# Autodesk Inventor assembly: axis5_6  compact
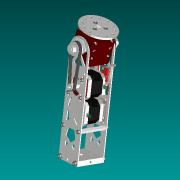
[picture p0: Inventor's stored thumbnail of the model, 180x180]
Saved by Autodesk Inventor 2020 (Build 240168000, 168)
## iProperties
Created: 2020-05-15
Part Number: axis5_6  compact
Document SubType Name: Assembly
Designer: stefa
Author: stefa
## Documents named in this file (21)
- D:\github_gedeeld\BeerMinder\3D-model\axis5_6\axis5_6  compact.iam
- D:\github_gedeeld\BeerMinder\3D-model\pulleys\GT2 Timing Pulley 36T - 8mm as.ipt
- D:\github_gedeeld\BeerMinder\3D-model\stepper motors\42BYG Stepper Motor.ipt
- D:\github_gedeeld\BeerMinder\3D-model\pulleys\GT2 Pulley 16T - 5mm as.ipt
- D:\github_gedeeld\BeerMinder\3D-model\axis5_6\bovenarm - links.ipt
- D:\github_gedeeld\BeerMinder\3D-model\bearings\lager 8mm - buiten 14 (sven 2 stuks).ipt
- D:\github_gedeeld\BeerMinder\3D-model\axis5_6\differential gearbox compact.iam
- D:\github_gedeeld\BeerMinder\3D-model\pulleys\tandriem32Tnaar16T_lengte280.ipt
- D:\github_gedeeld\BeerMinder\3D-model\pulleys\tandriem32Tnaar16T_lengte188.ipt
- D:\github_gedeeld\BeerMinder\3D-model\axis5_6\bovenarm - rechts.ipt
- D:\github_gedeeld\BeerMinder\3D-model\axis5_6\vul as platen.ipt
- D:\github_gedeeld\BeerMinder\3D-model\axis5_6\upvulling steppers axis5_6.ipt
- D:\github_gedeeld\BeerMinder\3D-model\boutjesEnMoertjes\ISO 4762 - M4 x 16ISO.ipt
- C:\Users\stefa\Documents\Inventor\Content Center Files\R2020\en-US\ISO 7089\ISO 7089 - 3 - 140 HV(1).ipt
- D:\github_gedeeld\BeerMinder\3D-model\axis5_6\bevestegingsKoppeling axis4_5.ipt
- C:\Users\stefa\Documents\Inventor\Content Center Files\R2020\en-US\ISO 7089\ISO 7089 - 4 - 140 HV(1).ipt
- C:\Users\stefa\Documents\Inventor\Content Center Files\R2020\en-US\ISO 4762(2)\ISO 4762 - M4 x 12ISO.ipt
- D:\github_gedeeld\BeerMinder\3D-model\axis5_6\lager opvulling voor lijm.ipt
- D:\github_gedeeld\BeerMinder\3D-model\boutjesEnMoertjes\ISO 4762 - M3 x 16ISO.ipt
- D:\github_gedeeld\BeerMinder\3D-model\ControlBox\swithces\Assembly - V-156-1C25 micro switch (Idle).iam
- D:\github_gedeeld\BeerMinder\3D-model\ControlBox\swithces\mini microswitchDM1-02P.iam
## Components (51 placed, 20 different names)
1. tandriem32Tnaar16T_lengte280:1 — Mate:57, Mate:58, Mate:139, Mate:143
2. tandriem32Tnaar16T_lengte188:1 — Mate:60, Mate:100, Mate:132, Mate:137
3. 42BYG Stepper Motor:2 — Tangent:120, Tangent:121, Mate:138, Mate:141, Angle:5, Mate:142
4. bovenarm - links:1 — Angle:3, Flush:6, Mate:113, Flush:14, Mate:118, Tangent:120, Tangent:121, Mate:123, Mate:124, Mate:134, Mate:140, Insert:4, Insert:5, Mate:156, Mate:158, Mate:160, Mate:162, Insert:20, Insert:22, Insert:23, Mate:198, Mate:200, Mate:204, Angle:6, Angle:7, Mate:205, Flush:16, Flush:17, Flush:19
5. GT2 Timing Pulley 36T - 8mm as:6 — Mate:57, Mate:58, Mate:115, Mate:134
6. GT2 Timing Pulley 36T - 8mm as:7 — Mate:60, Mate:100, Mate:114, Mate:133
7. bovenarm - rechts:1 — Flush:6, Mate:112, Flush:13, Mate:117, Tangent:122, Tangent:123, Mate:126, Mate:127, Mate:130, Mate:133, Insert:2, Insert:3, Mate:164, Mate:166, Mate:168, Mate:170, Mate:193, Mate:194, Insert:19, Mate:196, Mate:197, Mate:201
8. 42BYG Stepper Motor:3 — Tangent:122, Tangent:123, Mate:131, Mate:135, Mate:136, Angle:4
9. lager 8mm - buiten 14 (sven 2 stuks):1 — Mate:112, Flush:13, Mate:119, Mate:195
10. lager 8mm - buiten 14 (sven 2 stuks):2 — Mate:113, Flush:14, Mate:116, Mate:199
11. differential gearbox compact:1 [sub-assembly] — Mate:114, Mate:115, Mate:116, Mate:117, Mate:118, Mate:119, Angle:7, Mate:206
12. vul as platen:2 — Mate:124, Mate:126
13. vul as platen:3 — Mate:123, Mate:127
14. upvulling steppers axis5_6:1 — Mate:130, Mate:135, Mate:136, Angle:4, Mate:163, Mate:165, Mate:167, Mate:169, Mate:171, Mate:173, Mate:175, Mate:177
15. upvulling steppers axis5_6:2 — Mate:140, Mate:141, Angle:5, Mate:142, Mate:155, Mate:157, Mate:159, Mate:161, Mate:179, Mate:181, Mate:183, Mate:185
16. GT2 Pulley 16T - 5mm as:4 — Mate:131, Mate:132, Mate:137
17. GT2 Pulley 16T - 5mm as:5 — Mate:138, Mate:139, Mate:143
18. bevestegingsKoppeling axis4_5:1 — Mate:201, Mate:202, Mate:203
19. lager opvulling voor lijm:1 — Mate:195, Mate:196, Mate:197
20. lager opvulling voor lijm:2 — Mate:198, Mate:199, Mate:200
21. Assembly - V-156-1C25 micro switch (Idle):1 [sub-assembly] — Mate:204, Angle:6, Angle:8, Flush:15, Flush:17, Flush:19
22. Assembly - V-156-1C25 micro switch (Idle):2 [sub-assembly] — Mate:205, Angle:8, Flush:15, Flush:16
23. mini microswitchDM1-02P:1 [sub-assembly] — Mate:206
24. ISO 7089 4:1 — Mate:193, Mate:194, Insert:26
25. ISO 7089 4:3 — Insert:19, Insert:28
26. ISO 7089 4:4 — Insert:20, Insert:25
27. ISO 7089 4:6 — Insert:22
28. ISO 4762 M4 x 12:1 — Insert:23, Mate:203
29. ISO 4762 M4 x 12:3 — Insert:25, Mate:202
30. ISO 4762 M4 x 12:4 — Insert:26
31. ISO 4762 M4 x 12:6 — Insert:28
32. ISO 4762 M3 x 16:2 — Mate:185, Mate:186
33. ISO 4762 M3 x 16:1 — Mate:183, Mate:184
34. ISO 4762 M3 x 16:3 — Mate:181, Mate:182
35. ISO 4762 M3 x 16:4 — Mate:179, Mate:180
36. ISO 4762 M3 x 16:5 — Mate:177, Mate:178
37. ISO 4762 M3 x 16:6 — Mate:175, Mate:176
38. ISO 4762 M3 x 16:7 — Mate:173, Mate:174
39. ISO 4762 M3 x 16:8 — Mate:171, Mate:172
40. ISO 7089 3:9 — Mate:169, Mate:170
41. ISO 7089 3:8 — Mate:167, Mate:168
42. ISO 7089 3:7 — Mate:165, Mate:166
43. ISO 7089 3:6 — Mate:163, Mate:164, Mate:172, Mate:174, Mate:176, Mate:178
44. ISO 7089 3:5 — Mate:161, Mate:162
45. ISO 7089 3:4 — Mate:159, Mate:160
46. ISO 7089 3:3 — Mate:157, Mate:158
47. ISO 7089 3:2 — Mate:155, Mate:156, Mate:180, Mate:182, Mate:184, Mate:186
48. ISO 4762 M4 x 16:4 — Insert:5
49. ISO 4762 M4 x 16:5 — Insert:4
50. ISO 4762 M4 x 16:6 — Insert:3
51. ISO 4762 M4 x 16:7 — Insert:2
## Relationships (104: Mate 76, Insert 11, Flush 7, Angle 6, Tangent 4)
- Angle:3 (0 deg): bovenarm - links:1
- Mate:57 (0.5 mm): tandriem32Tnaar16T_lengte280:1 ↔ GT2 Timing Pulley 36T - 8mm as:6
- Mate:58: tandriem32Tnaar16T_lengte280:1 ↔ GT2 Timing Pulley 36T - 8mm as:6
- Mate:60 (0.5 mm): tandriem32Tnaar16T_lengte188:1 ↔ GT2 Timing Pulley 36T - 8mm as:7
- Flush:6: bovenarm - links:1 ↔ bovenarm - rechts:1
- Mate:100: tandriem32Tnaar16T_lengte188:1 ↔ GT2 Timing Pulley 36T - 8mm as:7
- Mate:112: bovenarm - rechts:1 ↔ lager 8mm - buiten 14 (sven 2 stuks):1
- Flush:13 (-2 mm): bovenarm - rechts:1 ↔ lager 8mm - buiten 14 (sven 2 stuks):1
- Mate:113: bovenarm - links:1 ↔ lager 8mm - buiten 14 (sven 2 stuks):2
- Flush:14 (-2 mm): bovenarm - links:1 ↔ lager 8mm - buiten 14 (sven 2 stuks):2
- Mate:114: GT2 Timing Pulley 36T - 8mm as:7 ↔ differential gearbox compact:1
- Mate:115: GT2 Timing Pulley 36T - 8mm as:6 ↔ differential gearbox compact:1
- Mate:116: lager 8mm - buiten 14 (sven 2 stuks):2 ↔ differential gearbox compact:1
- Mate:117 (1 mm): bovenarm - rechts:1 ↔ differential gearbox compact:1
- Mate:118 (1 mm): bovenarm - links:1 ↔ differential gearbox compact:1
- Tangent:120 (0.3 mm): 42BYG Stepper Motor:2 ↔ bovenarm - links:1
- Tangent:121 (0.3 mm): 42BYG Stepper Motor:2 ↔ bovenarm - links:1
- Mate:119: lager 8mm - buiten 14 (sven 2 stuks):1 ↔ differential gearbox compact:1
- Tangent:122 (0.3 mm): bovenarm - rechts:1 ↔ 42BYG Stepper Motor:3
- Tangent:123 (0.3 mm): bovenarm - rechts:1 ↔ 42BYG Stepper Motor:3
- Mate:123: bovenarm - links:1 ↔ vul as platen:3
- Mate:124: bovenarm - links:1 ↔ vul as platen:2
- Mate:126: bovenarm - rechts:1 ↔ vul as platen:2
- Mate:127: bovenarm - rechts:1 ↔ vul as platen:3
- Mate:130: bovenarm - rechts:1 ↔ upvulling steppers axis5_6:1
- Mate:131: 42BYG Stepper Motor:3 ↔ GT2 Pulley 16T - 5mm as:4
- Mate:132 (0.5 mm): tandriem32Tnaar16T_lengte188:1 ↔ GT2 Pulley 16T - 5mm as:4
- Mate:133 (3 mm): GT2 Timing Pulley 36T - 8mm as:7 ↔ bovenarm - rechts:1
- Mate:134 (3 mm): bovenarm - links:1 ↔ GT2 Timing Pulley 36T - 8mm as:6
- Mate:135: 42BYG Stepper Motor:3 ↔ upvulling steppers axis5_6:1
- Mate:136: 42BYG Stepper Motor:3 ↔ upvulling steppers axis5_6:1
- Angle:4 (0 deg): 42BYG Stepper Motor:3 ↔ upvulling steppers axis5_6:1
- Mate:137: tandriem32Tnaar16T_lengte188:1 ↔ GT2 Pulley 16T - 5mm as:4
- Mate:138: 42BYG Stepper Motor:2 ↔ GT2 Pulley 16T - 5mm as:5
- Mate:139 (0.5 mm): tandriem32Tnaar16T_lengte280:1 ↔ GT2 Pulley 16T - 5mm as:5
- Mate:140: bovenarm - links:1 ↔ upvulling steppers axis5_6:2
- Mate:141: 42BYG Stepper Motor:2 ↔ upvulling steppers axis5_6:2
- Angle:5 (0 deg): 42BYG Stepper Motor:2 ↔ upvulling steppers axis5_6:2
- Mate:142: 42BYG Stepper Motor:2 ↔ upvulling steppers axis5_6:2
- Mate:143: tandriem32Tnaar16T_lengte280:1 ↔ GT2 Pulley 16T - 5mm as:5
- Insert:2: bovenarm - rechts:1 ↔ ISO 4762 M4 x 16:7
- Insert:3: bovenarm - rechts:1 ↔ ISO 4762 M4 x 16:6
- Insert:4: bovenarm - links:1 ↔ ISO 4762 M4 x 16:5
- Insert:5: bovenarm - links:1 ↔ ISO 4762 M4 x 16:4
- Mate:155: upvulling steppers axis5_6:2 ↔ ISO 7089 3:2
- Mate:156: bovenarm - links:1 ↔ ISO 7089 3:2
- Mate:157: upvulling steppers axis5_6:2 ↔ ISO 7089 3:3
- Mate:158: bovenarm - links:1 ↔ ISO 7089 3:3
- Mate:159: upvulling steppers axis5_6:2 ↔ ISO 7089 3:4
- Mate:160: bovenarm - links:1 ↔ ISO 7089 3:4
- Mate:161: upvulling steppers axis5_6:2 ↔ ISO 7089 3:5
- Mate:162: bovenarm - links:1 ↔ ISO 7089 3:5
- Mate:163: upvulling steppers axis5_6:1 ↔ ISO 7089 3:6
- Mate:164: bovenarm - rechts:1 ↔ ISO 7089 3:6
- Mate:165: upvulling steppers axis5_6:1 ↔ ISO 7089 3:7
- Mate:166: bovenarm - rechts:1 ↔ ISO 7089 3:7
- Mate:167: upvulling steppers axis5_6:1 ↔ ISO 7089 3:8
- Mate:168: bovenarm - rechts:1 ↔ ISO 7089 3:8
- Mate:169: upvulling steppers axis5_6:1 ↔ ISO 7089 3:9
- Mate:170: bovenarm - rechts:1 ↔ ISO 7089 3:9
- Mate:171: upvulling steppers axis5_6:1 ↔ ISO 4762 M3 x 16:8
- Mate:172: ISO 4762 M3 x 16:8 ↔ ISO 7089 3:6
- Mate:173: upvulling steppers axis5_6:1 ↔ ISO 4762 M3 x 16:7
- Mate:174: ISO 4762 M3 x 16:7 ↔ ISO 7089 3:6
- Mate:175: upvulling steppers axis5_6:1 ↔ ISO 4762 M3 x 16:6
- Mate:176: ISO 4762 M3 x 16:6 ↔ ISO 7089 3:6
- Mate:177: upvulling steppers axis5_6:1 ↔ ISO 4762 M3 x 16:5
- Mate:178: ISO 4762 M3 x 16:5 ↔ ISO 7089 3:6
- Mate:179: upvulling steppers axis5_6:2 ↔ ISO 4762 M3 x 16:4
- Mate:180: ISO 4762 M3 x 16:4 ↔ ISO 7089 3:2
- Mate:181: upvulling steppers axis5_6:2 ↔ ISO 4762 M3 x 16:3
- Mate:182: ISO 4762 M3 x 16:3 ↔ ISO 7089 3:2
- Mate:183: upvulling steppers axis5_6:2 ↔ ISO 4762 M3 x 16:1
- Mate:184: ISO 4762 M3 x 16:1 ↔ ISO 7089 3:2
- Mate:185: upvulling steppers axis5_6:2 ↔ ISO 4762 M3 x 16:2
- Mate:186: ISO 4762 M3 x 16:2 ↔ ISO 7089 3:2
- Mate:193: bovenarm - rechts:1 ↔ ISO 7089 4:1
- Mate:194: bovenarm - rechts:1 ↔ ISO 7089 4:1
- Insert:19: bovenarm - rechts:1 ↔ ISO 7089 4:3
- Insert:20: bovenarm - links:1 ↔ ISO 7089 4:4
- Insert:22: bovenarm - links:1 ↔ ISO 7089 4:6
- Insert:23: bovenarm - links:1 ↔ ISO 4762 M4 x 12:1
- Insert:25: ISO 7089 4:4 ↔ ISO 4762 M4 x 12:3
- Insert:26: ISO 7089 4:1 ↔ ISO 4762 M4 x 12:4
- Insert:28: ISO 7089 4:3 ↔ ISO 4762 M4 x 12:6
- Mate:195: lager 8mm - buiten 14 (sven 2 stuks):1 ↔ lager opvulling voor lijm:1
- Mate:196: bovenarm - rechts:1 ↔ lager opvulling voor lijm:1
- Mate:197: bovenarm - rechts:1 ↔ lager opvulling voor lijm:1
- Mate:198: bovenarm - links:1 ↔ lager opvulling voor lijm:2
- Mate:199: lager 8mm - buiten 14 (sven 2 stuks):2 ↔ lager opvulling voor lijm:2
- Mate:200: bovenarm - links:1 ↔ lager opvulling voor lijm:2
- Mate:201: bovenarm - rechts:1 ↔ bevestegingsKoppeling axis4_5:1
- Mate:202: bevestegingsKoppeling axis4_5:1 ↔ ISO 4762 M4 x 12:3
- Mate:203: bevestegingsKoppeling axis4_5:1 ↔ ISO 4762 M4 x 12:1
- Mate:204: bovenarm - links:1 ↔ Assembly - V-156-1C25 micro switch (Idle):1
- Angle:6 (0 deg): bovenarm - links:1 ↔ Assembly - V-156-1C25 micro switch (Idle):1
- Angle:7 (180 deg): bovenarm - links:1 ↔ differential gearbox compact:1
- Mate:205: bovenarm - links:1 ↔ Assembly - V-156-1C25 micro switch (Idle):2
- Angle:8 (0 deg): Assembly - V-156-1C25 micro switch (Idle):1 ↔ Assembly - V-156-1C25 micro switch (Idle):2
- Flush:15: Assembly - V-156-1C25 micro switch (Idle):1 ↔ Assembly - V-156-1C25 micro switch (Idle):2
- Flush:16: bovenarm - links:1 ↔ Assembly - V-156-1C25 micro switch (Idle):2
- Flush:17: bovenarm - links:1 ↔ Assembly - V-156-1C25 micro switch (Idle):1
- Flush:19: bovenarm - links:1 ↔ Assembly - V-156-1C25 micro switch (Idle):1
- Mate:206: differential gearbox compact:1 ↔ mini microswitchDM1-02P:1
